# Autodesk Inventor assembly: FInal Cover Assembly
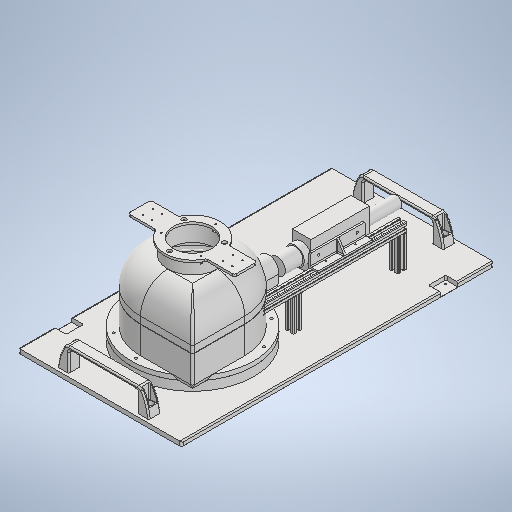
[picture p0: Inventor's stored thumbnail of the model, 512x512]
Saved by Autodesk Inventor 2025 (Build 290162000, 162)
## iProperties
Created: 2025-10-13
Part Number: FInal Cover Assembly
Document SubType Name: Assembly
Designer: mumin
Author: mumin
## Documents named in this file (14)
- C:\GitHub\In-situ-monitoring-of-powder-bed-fusion-additive-manufacturing\system_development\Orichalcum\v0.3\FInal Cover Assembly.iam
- C:\GitHub\In-situ-monitoring-of-powder-bed-fusion-additive-manufacturing\system_development\Orichalcum\v0.3\12mm Cover.ipt
- C:\GitHub\In-situ-monitoring-of-powder-bed-fusion-additive-manufacturing\system_development\Orichalcum\v0.3\SealedGlassRing.ipt
- C:\GitHub\In-situ-monitoring-of-powder-bed-fusion-additive-manufacturing\system_development\Orichalcum\v0.3\Cylinder Housing_base_3.ipt
- C:\GitHub\In-situ-monitoring-of-powder-bed-fusion-additive-manufacturing\system_development\Orichalcum\v0.3\Cylinder Housing_cap_3.ipt
- C:\GitHub\In-situ-monitoring-of-powder-bed-fusion-additive-manufacturing\system_development\Orichalcum\v0.3\2020 Legs (70mm).ipt
- C:\GitHub\In-situ-monitoring-of-powder-bed-fusion-additive-manufacturing\system_development\Orichalcum\v0.3\2020 LV-GVS Beam (481).ipt
- C:\GitHub\In-situ-monitoring-of-powder-bed-fusion-additive-manufacturing\system_development\Orichalcum\v0.3\GVS_Plate.ipt
- C:\GitHub\In-situ-monitoring-of-powder-bed-fusion-additive-manufacturing\system_development\Orichalcum\v0.3\GVS102-Step.ipt
- C:\GitHub\In-situ-monitoring-of-powder-bed-fusion-additive-manufacturing\system_development\Orichalcum\v0.3\CenterCylinder_2.ipt
- C:\GitHub\In-situ-monitoring-of-powder-bed-fusion-additive-manufacturing\system_development\Orichalcum\v0.3\LV_Bracket_2.ipt
- C:\GitHub\In-situ-monitoring-of-powder-bed-fusion-additive-manufacturing\system_development\Orichalcum\v0.3\Handle.ipt
- C:\GitHub\In-situ-monitoring-of-powder-bed-fusion-additive-manufacturing\system_development\Orichalcum\v0.3\Updated Laser Scanner.ipt
- C:\GitHub\In-situ-monitoring-of-powder-bed-fusion-additive-manufacturing\system_development\Orichalcum\v0.3\Metal Head Plate.ipt
## Components (15 placed, 13 different names)
1. 12mm Cover:1 — Insert:1, Insert:2, Insert:5, Insert:8, Insert:9, Insert:10
2. SealedGlassRing:1 — Insert:1, Insert:2, Insert:3, Insert:4
3. Cylinder Housing_base_3:1 — Insert:3, Insert:4, Mate:1, Flush:1, Flush:2
4. Cylinder Housing_cap_3:1 — Mate:1, Flush:1, Flush:2, Mate:4
5. 2020 Legs (70mm):1 — Insert:5, Flush:3, Mate:2, Flush:4
6. 2020 LV-GVS Beam (481):1 — Flush:3, Mate:2, Flush:4, Flush:5, Mate:3, Mate:5, Flush:6
7. GVS_Plate:1 — Flush:5, Mate:3, Insert:6, Insert:7
8. GVS102-Step:1 — Insert:6, Insert:7
9. CenterCylinder_2:1 — Mate:4, Insert:13, Insert:14
10. 2020 Legs (70mm):2 — Insert:8
11. LV_Bracket_2:1 — Mate:5, Flush:6, Insert:11, Insert:12
12. Handle:1 — Insert:9
13. Handle:2 — Insert:10
14. Updated Laser Scanner:1 — Insert:11, Insert:12
15. Metal Head Plate:1 — Insert:13, Insert:14
## Relationships (25: Insert 14, Flush 6, Mate 5)
- Insert:1: 12mm Cover:1 ↔ SealedGlassRing:1
- Insert:2: 12mm Cover:1 ↔ SealedGlassRing:1
- Insert:3: SealedGlassRing:1 ↔ Cylinder Housing_base_3:1
- Insert:4: SealedGlassRing:1 ↔ Cylinder Housing_base_3:1
- Mate:1: Cylinder Housing_base_3:1 ↔ Cylinder Housing_cap_3:1
- Flush:1: Cylinder Housing_base_3:1 ↔ Cylinder Housing_cap_3:1
- Flush:2: Cylinder Housing_base_3:1 ↔ Cylinder Housing_cap_3:1
- Insert:5: 12mm Cover:1 ↔ 2020 Legs (70mm):1
- Flush:3: 2020 Legs (70mm):1 ↔ 2020 LV-GVS Beam (481):1
- Mate:2: 2020 Legs (70mm):1 ↔ 2020 LV-GVS Beam (481):1
- Flush:4: 2020 Legs (70mm):1 ↔ 2020 LV-GVS Beam (481):1
- Flush:5: 2020 LV-GVS Beam (481):1 ↔ GVS_Plate:1
- Mate:3: 2020 LV-GVS Beam (481):1 ↔ GVS_Plate:1
- Insert:6: GVS_Plate:1 ↔ GVS102-Step:1
- Insert:7: GVS_Plate:1 ↔ GVS102-Step:1
- Mate:4: Cylinder Housing_cap_3:1 ↔ CenterCylinder_2:1
- Insert:8: 12mm Cover:1 ↔ 2020 Legs (70mm):2
- Mate:5: 2020 LV-GVS Beam (481):1 ↔ LV_Bracket_2:1
- Flush:6: 2020 LV-GVS Beam (481):1 ↔ LV_Bracket_2:1
- Insert:9: 12mm Cover:1 ↔ Handle:1
- Insert:10: 12mm Cover:1 ↔ Handle:2
- Insert:11: LV_Bracket_2:1 ↔ Updated Laser Scanner:1
- Insert:12: LV_Bracket_2:1 ↔ Updated Laser Scanner:1
- Insert:13: CenterCylinder_2:1 ↔ Metal Head Plate:1
- Insert:14: CenterCylinder_2:1 ↔ Metal Head Plate:1
